# Autodesk Inventor assembly: AnalogClock
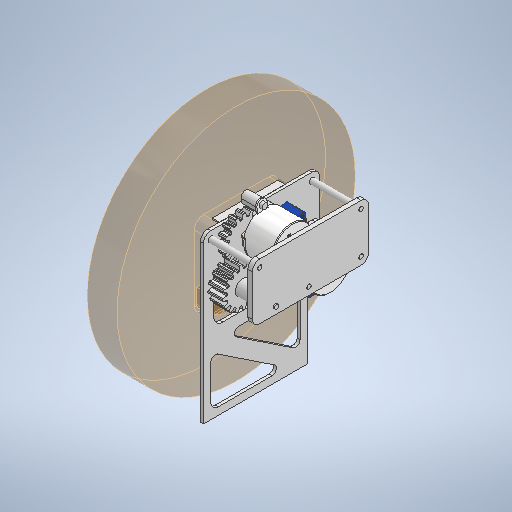
[picture p0: Inventor's stored thumbnail of the model, 512x512]
Saved by Autodesk Inventor 2025.2 (Build 292293000, 293)
## iProperties
Created: 2026-02-21
Part Number: AnalogClock
Document SubType Name: Assembly
Designer: naka6
Author: naka6
## iProperties of the stored document Step - 28BYJ-48.ipt
Created: 2020-05-16
Part Number: Step - 28BYJ-48
Material: 一般
Document SubType Name: Modeling
Designer: naka6
Density: 1 g/cm^3
Appearance: 既定
Sending System: SolidWorks 2017
Last Author: bbayl
Last Saved: 2020-05-16
Author: naka6
## Documents named in this file (10)
- C:\Users\naka6\Projects\TimeFaker\AnalogClock.iam
- C:\Users\naka6\Projects\TimeFaker\Clack.ipt
- **C:\Users\naka6\Projects\TimeFaker\AnalogClock.iam*LocalDocs*xAaaaauaaAaaaaaaaAaaaqbbfBf*Step - 28BYJ-48.ipt
- C:\Users\naka6\Projects\TimeFaker\base.ipt
- C:\Users\naka6\Projects\TimeFaker\CaseBase.ipt
- C:\Users\naka6\Projects\TimeFaker\GearDirect.ipt
- C:\Users\naka6\Projects\TimeFaker\GearMotor.ipt
- C:\Users\naka6\Projects\TimeFaker\Jig.ipt
- C:\Users\naka6\Projects\TimeFaker\CaseCover.ipt
- C:\Users\naka6\Projects\TimeFaker\rohs-step-motor-28byj-48-1.snapshot.5\Step - 28BYJ-48.SLDPRT
## Components (9 placed, 8 different names)
1. Clack:1 — 角度:2, フラッシュ:1, フラッシュ:2, フラッシュ:3
2. Step - 28BYJ-48:1 — 角度:2, メイト:1, メイト:2, メイト:5, フラッシュ:5, 挿入:2, フラッシュ:6
3. Step - 28BYJ-48:2 — メイト:4, フラッシュ:4, 挿入:1, 挿入:3
4. base:1 — フラッシュ:1
5. CaseBase:1 — フラッシュ:2, メイト:1, メイト:2, 挿入:2
6. GearDirect:1 — フラッシュ:3
7. GearMotor:1 — メイト:4, フラッシュ:4
8. Jig:1 — メイト:5, フラッシュ:5, 挿入:1, 挿入:3
9. CaseCover:1 — フラッシュ:6
## Relationships (14: Flush 6, Mate 4, Insert 3, Angle 1)
- 角度:2 [Angle] (0 deg): Clack:1 ↔ Step - 28BYJ-48:1
- フラッシュ:1 [Flush]: Clack:1 ↔ base:1
- フラッシュ:2 [Flush]: Clack:1 ↔ CaseBase:1
- メイト:1 [Mate]: Step - 28BYJ-48:1 ↔ CaseBase:1
- メイト:2 [Mate]: Step - 28BYJ-48:1 ↔ CaseBase:1
- フラッシュ:3 [Flush]: Clack:1 ↔ GearDirect:1
- メイト:4 [Mate]: Step - 28BYJ-48:2 ↔ GearMotor:1
- フラッシュ:4 [Flush]: Step - 28BYJ-48:2 ↔ GearMotor:1
- メイト:5 [Mate]: Step - 28BYJ-48:1 ↔ Jig:1
- フラッシュ:5 [Flush]: Step - 28BYJ-48:1 ↔ Jig:1
- 挿入:1 [Insert]: Step - 28BYJ-48:2 ↔ Jig:1
- 挿入:2 [Insert]: Step - 28BYJ-48:1 ↔ CaseBase:1
- 挿入:3 [Insert]: Step - 28BYJ-48:2 ↔ Jig:1
- フラッシュ:6 [Flush]: Step - 28BYJ-48:1 ↔ CaseCover:1
